# Autodesk Inventor assembly: McCrea_head_walle
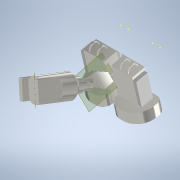
[picture p0: Inventor's stored thumbnail of the model, 180x180]
Saved by Autodesk Inventor 2022 (Build 260153000, 153)
## iProperties
Created: 2022-01-20
Part Number: McCrea_head_walle
Document SubType Name: Assembly
Designer: MatusBarany
Author: MatusBarany
## Documents named in this file (20)
- C:\Users\Max\Documents\Škola\teg\wall-e\assembly\McCrea_head_walle.iam
- C:\Users\Max\Documents\Škola\teg\wall-e\maxo\McCrea_kabel_walle.ipt
- C:\Users\Max\Documents\Škola\teg\wall-e\maxo\McCrea_krk_walle.ipt
- C:\Users\Max\Documents\Škola\teg\wall-e\maxo\McCrea_oblucik_walle.ipt
- C:\Users\Max\Documents\Škola\teg\wall-e\maxo\McCrea_oko_walle.ipt
- C:\Users\Max\Documents\Škola\teg\wall-e\maxo\McCrea_palicka_walle.ipt
- C:\Users\Max\Documents\Škola\teg\wall-e\maxo\McCrea_uhco_walle.ipt
- C:\Users\Max\Documents\Škola\teg\wall-e\maxo\McCrea_velka_palicka_walle.ipt
- C:\Users\Max\Documents\Škola\teg\wall-e\maxo\McCrea_velka_palicka_walle_1.ipt
- C:\Users\Max\Documents\Škola\teg\wall-e\maxo\McCrea_velky_krk_walle.ipt
- C:\Users\Max\Documents\Škola\teg\wall-e\maxo\McCrea_zadna_cast_oka_walle.ipt
- C:\Users\Max\Documents\Škola\teg\wall-e\maxo\McCrea_zadne_oko_walle.ipt
- C:\Users\Max\Documents\Škola\teg\wall-e\maxo\McCrea_doska_walle.ipt
- C:\Users\Max\Documents\Škola\teg\wall-e\maxo\McCrea_uhco_walle_MIR1.ipt
- C:\Users\Max\Documents\Škola\teg\wall-e\maxo\McCrea_zadna_cast_oka_walle_MIR1.ipt
- C:\Users\Max\Documents\Škola\teg\wall-e\maxo\McCrea_kabel_walle_MIR1.ipt
- C:\Users\Max\Documents\Škola\teg\wall-e\maxo\McCrea_oko_walle_MIR1.ipt
- C:\Users\Max\Documents\Škola\teg\wall-e\maxo\McCrea_velka_palicka_walle_MIR1.ipt
- C:\Users\Max\Documents\Škola\teg\wall-e\maxo\McCrea_zadne_oko_walle_MIR1.ipt
- C:\Users\Max\Documents\Škola\teg\wall-e\maxo\McCrea_doska_walle_MIR.ipt
## Components (23 placed, 19 different names)
1. McCrea_krk_walle:1 — Rigid:1, Rigid:2, Insert:2
2. McCrea_oblucik_walle:1 — Rotational:2, Rigid:2
3. McCrea_palicka_walle:1 — Rotational:1
4. McCrea_uhco_walle:1 — Mate:2, Flush:1
5. McCrea_zadna_cast_oka_walle:1 — Rigid:3, Mate:1, Flush:3
6. McCrea_kabel_walle:2 — Mate:3
7. McCrea_oblucik_walle:2 — Rotational:1, Rigid:1
8. McCrea_oko_walle:2 — Rigid:3, Cylindrical:1, Flush:4
9. McCrea_palicka_walle:2 — Rotational:2
10. McCrea_velka_palicka_walle:2 — Cylindrical:1, Flush:4
11. McCrea_velka_palicka_walle_1:2 — Rotational:4, Insert:1
12. McCrea_velky_krk_walle:2 — Insert:1, Flush:2, Insert:2
13. McCrea_zadne_oko_walle:2 — Mate:1, Mate:2, Flush:1, Mate:3, Mate:4, Mate:5, Mate:12, Flush:3
14. McCrea_kabel_walle:3 — Mate:4
15. McCrea_doska_walle:1 — Mate:5, Rotational:4, Mate:12
16. McCrea_uhco_walle_MIR1:1 — Flush:7, Mate:14
17. McCrea_zadna_cast_oka_walle_MIR1:1 — Flush:6, Mate:15, Rigid:4
18. McCrea_kabel_walle_MIR1:1 — Mate:13
19. McCrea_oko_walle_MIR1:1 — Flush:5, Rigid:4, Cylindrical:2
20. McCrea_velka_palicka_walle_MIR1:1 — Flush:5, Cylindrical:2
21. McCrea_zadne_oko_walle_MIR1:1 — Flush:6, Mate:13, Flush:7, Mate:14, Mate:15, Mate:16, Mate:17, Mate:18
22. McCrea_kabel_walle_MIR1:2 — Mate:16
23. McCrea_doska_walle_MIR:1 — Mate:17, Mate:18
## Relationships (30: Mate 12, Flush 7, WeldJoint 4, RevoluteJoint 3, Insert 2, CylindricalJoint 2)
- Rotational:1 [RevoluteJoint]: McCrea_palicka_walle:1 ↔ McCrea_oblucik_walle:2
- Rigid:1 [WeldJoint]: McCrea_krk_walle:1 ↔ McCrea_oblucik_walle:2
- Rotational:2 [RevoluteJoint]: McCrea_oblucik_walle:1 ↔ McCrea_palicka_walle:2
- Rigid:2 [WeldJoint]: McCrea_krk_walle:1 ↔ McCrea_oblucik_walle:1
- Rigid:3 [WeldJoint]: McCrea_zadna_cast_oka_walle:1 ↔ McCrea_oko_walle:2
- Mate:1: McCrea_zadna_cast_oka_walle:1 ↔ McCrea_zadne_oko_walle:2
- Mate:2: McCrea_uhco_walle:1 ↔ McCrea_zadne_oko_walle:2
- Flush:1: McCrea_uhco_walle:1 ↔ McCrea_zadne_oko_walle:2
- Mate:3: McCrea_kabel_walle:2 ↔ McCrea_zadne_oko_walle:2
- Mate:4: McCrea_zadne_oko_walle:2 ↔ McCrea_kabel_walle:3
- Mate:5: McCrea_zadne_oko_walle:2 ↔ McCrea_doska_walle:1
- Rotational:4 [RevoluteJoint]: McCrea_velka_palicka_walle_1:2 ↔ McCrea_doska_walle:1
- Insert:1: McCrea_velka_palicka_walle_1:2 ↔ McCrea_velky_krk_walle:2
- Flush:2 (-3.5 mm): McCrea_velky_krk_walle:2
- Mate:12: McCrea_zadne_oko_walle:2 ↔ McCrea_doska_walle:1
- Flush:3: McCrea_zadna_cast_oka_walle:1 ↔ McCrea_zadne_oko_walle:2
- Cylindrical:1: McCrea_oko_walle:2 ↔ McCrea_velka_palicka_walle:2
- Flush:4: McCrea_oko_walle:2 ↔ McCrea_velka_palicka_walle:2
- Flush:5: McCrea_oko_walle_MIR1:1 ↔ McCrea_velka_palicka_walle_MIR1:1
- Flush:6: McCrea_zadna_cast_oka_walle_MIR1:1 ↔ McCrea_zadne_oko_walle_MIR1:1
- Mate:13: McCrea_kabel_walle_MIR1:1 ↔ McCrea_zadne_oko_walle_MIR1:1
- Flush:7: McCrea_uhco_walle_MIR1:1 ↔ McCrea_zadne_oko_walle_MIR1:1
- Mate:14: McCrea_uhco_walle_MIR1:1 ↔ McCrea_zadne_oko_walle_MIR1:1
- Mate:15: McCrea_zadna_cast_oka_walle_MIR1:1 ↔ McCrea_zadne_oko_walle_MIR1:1
- Mate:16: McCrea_zadne_oko_walle_MIR1:1 ↔ McCrea_kabel_walle_MIR1:2
- Mate:17: McCrea_zadne_oko_walle_MIR1:1 ↔ McCrea_doska_walle_MIR:1
- Mate:18: McCrea_zadne_oko_walle_MIR1:1 ↔ McCrea_doska_walle_MIR:1
- Rigid:4 [WeldJoint]: McCrea_zadna_cast_oka_walle_MIR1:1 ↔ McCrea_oko_walle_MIR1:1
- Cylindrical:2: McCrea_oko_walle_MIR1:1 ↔ McCrea_velka_palicka_walle_MIR1:1
- Insert:2: McCrea_krk_walle:1 ↔ McCrea_velky_krk_walle:2
